# Autodesk Inventor assembly: chaimber
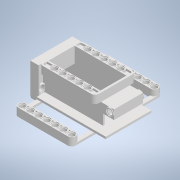
[picture p0: Inventor's stored thumbnail of the model, 180x180]
Saved by Autodesk Inventor 2021 (Build 250183000, 183)
## iProperties
Created: 2024-03-19
Part Number: chaimber
Document SubType Name: Assembly
Designer: 22hamfri
Author: 22hamfri
## Documents named in this file (5)
- C:\Users\22hamfri\Documents\School\Programmering\domino\chaimber.iam
- C:\Users\22hamfri\Documents\School\Programmering\domino\chaimber-adapter.ipt
- C:\Users\22hamfri\Documents\School\Programmering\domino\chaimber.ipt
- C:\Users\22hamfri\Documents\School\Programmering\domino\magazine-adapter.ipt
- C:\Users\22hamfri\Documents\School\Programmering\domino\battery-adapter.ipt
## Components (4 placed, 4 different names)
1. chaimber-adapter:1 — Rigid:1
2. chaimber:1 — Rigid:1, Rigid:3, Rigid:4
3. magazine-adapter:1 — Rigid:3
4. battery-adapter:1 — Rigid:4
## Relationships (3: WeldJoint 3)
- Rigid:1 [WeldJoint]: chaimber-adapter:1 ↔ chaimber:1
- Rigid:3 [WeldJoint]: chaimber:1 ↔ magazine-adapter:1
- Rigid:4 [WeldJoint]: chaimber:1 ↔ battery-adapter:1
